# Autodesk Inventor assembly: bett_V3_doppelt1
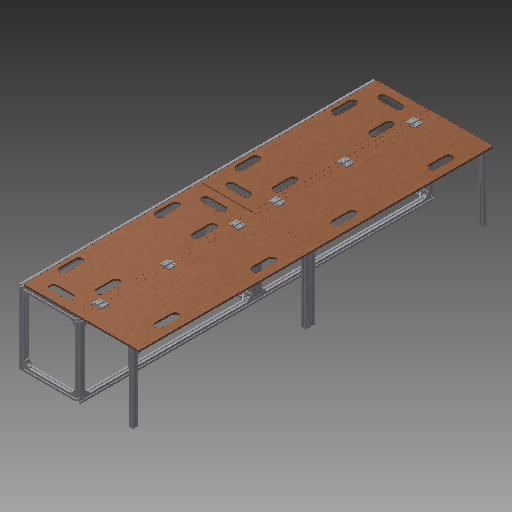
[picture p0: Inventor's stored thumbnail of the model, 512x512]
Saved by Autodesk Inventor 2018 (Build 220112000, 112)
## iProperties
Created: 2020-04-19
Part Number: bett_V3_doppelt1
Material: Generisch
Document SubType Name: Assembly
Designer: wepet
Author: wepet
## Documents named in this file (5)
- C:\Users\wepet\Downloads\anhaenger\current\details\bett\bett_V3\bett_V3_doppelt1.iam
- C:\Users\wepet\Downloads\anhaenger\current\details\bett\bett_V3\bett_V3_teil4_bein.iam
- C:\Users\wepet\Downloads\anhaenger\current\details\bett\bett_V3\bett_V3_teil2_deckplatte_skizze.ipt
- C:\Users\wepet\Downloads\anhaenger\current\details\bett\bett_V3\bett_V3_teil3_klappe.iam
- C:\Users\wepet\Downloads\anhaenger\current\details\bett\bett_V3\bett_V3_teil1_sitzbank.iam
## Components (10 placed, 4 different names)
1. bett_V3_teil1_sitzbank:1 [sub-assembly] — Passend:1, Passend:2, Passend:3, Drehbar:5, Fluchtend:1, Drehbar:6, Passend:4, Fluchtend:3, Fluchtend:4
2. bett_V3_teil2_deckplatte_skizze:1 — Fluchtend:1, Drehbar:6
3. bett_V3_teil3_klappe:1 [sub-assembly] — Drehbar:3, Drehbar:4, Drehbar:5
4. bett_V3_teil4_bein:1 [sub-assembly] — Drehbar:3
5. bett_V3_teil4_bein:2 [sub-assembly] — Drehbar:4
6. bett_V3_teil4_bein:3 [sub-assembly] — Drehbar:7
7. bett_V3_teil2_deckplatte_skizze:2
8. bett_V3_teil3_klappe:2 [sub-assembly] — Drehbar:7, Drehbar:8
9. bett_V3_teil1_sitzbank:2 [sub-assembly] — Passend:4, Fluchtend:3, Fluchtend:4
10. bett_V3_teil4_bein:4 [sub-assembly] — Drehbar:8
## Relationships (16: RevoluteJoint 8, Mate 4, Flush 4)
- Passend:1 [Mate]: bett_V3_teil1_sitzbank:1
- Passend:2 [Mate]: bett_V3_teil1_sitzbank:1
- Passend:3 [Mate]: bett_V3_teil1_sitzbank:1
- Drehbar:3 [RevoluteJoint]: bett_V3_teil3_klappe:1 ↔ bett_V3_teil4_bein:1
- Drehbar:4 [RevoluteJoint]: bett_V3_teil3_klappe:1 ↔ bett_V3_teil4_bein:2
- Drehbar:5 [RevoluteJoint]: bett_V3_teil1_sitzbank:1 ↔ bett_V3_teil3_klappe:1
- Fluchtend:1 [Flush]: bett_V3_teil1_sitzbank:1 ↔ bett_V3_teil2_deckplatte_skizze:1
- Drehbar:6 [RevoluteJoint]: bett_V3_teil1_sitzbank:1 ↔ bett_V3_teil2_deckplatte_skizze:1
- Drehbar:7 [RevoluteJoint]: bett_V3_teil4_bein:3 ↔ bett_V3_teil3_klappe:2
- Drehbar:8 [RevoluteJoint]: bett_V3_teil3_klappe:2 ↔ bett_V3_teil4_bein:4
- [RevoluteJoint]: bett_V3_teil3_klappe:2 ↔ bett_V3_teil1_sitzbank:2
- [Flush]: bett_V3_teil2_deckplatte_skizze:2 ↔ bett_V3_teil1_sitzbank:2
- [RevoluteJoint]: bett_V3_teil2_deckplatte_skizze:2 ↔ bett_V3_teil1_sitzbank:2
- Passend:4 [Mate]: bett_V3_teil1_sitzbank:1 ↔ bett_V3_teil1_sitzbank:2
- Fluchtend:3 [Flush]: bett_V3_teil1_sitzbank:1 ↔ bett_V3_teil1_sitzbank:2
- Fluchtend:4 [Flush]: bett_V3_teil1_sitzbank:1 ↔ bett_V3_teil1_sitzbank:2
## Named parameters: d36_d12 = 0 mm, d37_d13 = -0.000001 deg, d38_d14 = 0 deg, d39_d15 = -90 deg, d40_d20 = 0 mm, d41_d21 = -152.631576 deg, d42_d22 = -152.63 deg, d43_d23 = -242.63 deg, d44_d27 = 0 mm, d45_d28 = 77.79 deg, d46_d29 = 77.79 deg, d47_d30 = -102.21 deg, d48_d31 = 0 mm, d49_d32 = 0 mm, d50_d33 = 179.889048 deg, d51_d34 = 180 deg, d52_d35 = 90 deg
